# Autodesk Inventor assembly: Robot_eslabones
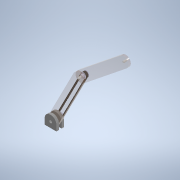
[picture p0: Inventor's stored thumbnail of the model, 180x180]
Saved by Autodesk Inventor 2021 (Build 250183000, 183)
## iProperties
Created: 2022-01-12
Part Number: Robot_eslabones
Document SubType Name: Assembly
Designer: Yeison
Author: Yeison
## Documents named in this file (7)
- C:\Users\Yeison\Documents\GitHub\Servomecanismos\Modelo 2021\Robot_eslabones.iam
- C:\Users\Yeison\Documents\GitHub\Servomecanismos\Modelo 2021\Soporte.ipt
- C:\Users\Yeison\Documents\GitHub\Servomecanismos\Modelo 2021\pin2.ipt
- C:\Users\Yeison\Documents\GitHub\Servomecanismos\Modelo 2021\Eslabon.ipt
- C:\Users\Yeison\Documents\GitHub\Servomecanismos\Modelo 2021\pin1.ipt
- C:\Users\Yeison\Documents\GitHub\Servomecanismos\Modelo 2021\Polea.ipt
- C:\Users\Yeison\Documents\GitHub\Servomecanismos\Modelo 2021\Correa.ipt
## Components (9 placed, 6 different names)
1. Soporte:1 — Rigid:4, Rigid:5
2. pin2:1 — Rotational:1, Rigid:4
3. Eslabon:1 — Rotational:1, Rigid:2
4. pin2:2 — Rigid:2, Rotational:2, Rotational:3
5. Eslabon:2 — Rotational:2, Rigid:3
6. pin1:1 — Rigid:3
7. Polea:1 — Rigid:5, Rotational:4
8. Polea:2 — Rotational:3, Rotational:5
9. Correa:1 — Rotational:4, Rotational:5
## Relationships (9: RevoluteJoint 5, WeldJoint 4)
- Rotational:1 [RevoluteJoint]: pin2:1 ↔ Eslabon:1
- Rigid:2 [WeldJoint]: Eslabon:1 ↔ pin2:2
- Rotational:2 [RevoluteJoint] (-10 mm): pin2:2 ↔ Eslabon:2
- Rigid:3 [WeldJoint]: Eslabon:2 ↔ pin1:1
- Rigid:4 [WeldJoint]: Soporte:1 ↔ pin2:1
- Rigid:5 [WeldJoint]: Soporte:1 ↔ Polea:1
- Rotational:3 [RevoluteJoint]: pin2:2 ↔ Polea:2
- Rotational:4 [RevoluteJoint]: Polea:1 ↔ Correa:1
- Rotational:5 [RevoluteJoint]: Polea:2 ↔ Correa:1
